# Autodesk Inventor assembly: Rotary_system_1
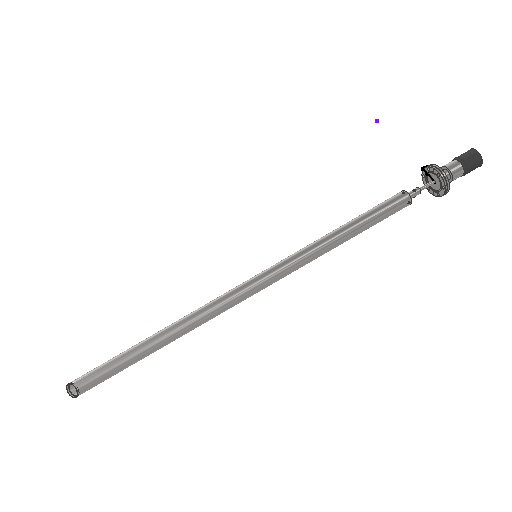
[picture p0: Inventor's stored thumbnail of the model, 512x512]
Saved by Autodesk Inventor 2026.2 (Build 302298000, 298)
## iProperties
Created: 2026-06-01
Part Number: Rotary_system_1
Document SubType Name: Assembly
Designer: zetsu
Author: zetsu
## Documents named in this file (7)
- D:\repos\PIHTI\BoronProbe_5\Figures\Rotary_system_1.iam
- D:\repos\PIHTI\BoronProbe_5\parts\B_probe_pipe_5.ipt
- D:\repos\PIHTI\BoronProbe_5\parts\rotary_transfer_shaft_5_1.ipt
- D:\repos\PIHTI\BoronProbe_5\parts\Rotary_Feedthrough\Rotary_Feedthrough.iam
- D:\repos\PIHTI\BoronProbe_5\parts\M3x10-BHCS.ipt
- D:\repos\PIHTI\BoronProbe_5\parts\M3x20-BHCS.ipt
- D:\repos\PIHTI\BoronProbe_5\parts\M3-nut.ipt
## Components (9 placed, 5 different names)
1. B_probe_pipe_5:1 — メイト:1, メイト:2, メイト:3, メイト:5, メイト:7, メイト:9
2. rotary_transfer_shaft_5_1:1 — メイト:1, メイト:2, メイト:4, メイト:6, メイト:8, メイト:10, メイト:11, メイト:12, メイト:13, メイト:14, メイト:15
3. Rotary_Feedthrough:1 [sub-assembly] — メイト:11, メイト:12
4. Broached Hexagon Socket Button Head Cap Screw - Metric M3 x 0.5 x 6:1 — メイト:3, メイト:4
5. Broached Hexagon Socket Button Head Cap Screw - Metric M3 x 0.5 x 6:2 — メイト:5, メイト:6
6. Broached Hexagon Socket Button Head Cap Screw - Metric M3 x 0.5 x 6:3 — メイト:7, メイト:8
7. Broached Hexagon Socket Button Head Cap Screw - Metric M3 x 0.5 x 6:4 — メイト:9, メイト:10
8. Broached Hexagon Socket Button Head Cap Screw - Metric M3 x 0.5 x 6:5 — メイト:13, メイト:14, メイト:16
9. JIS B 1181 Style 1 - Metric A M3:1 — メイト:15, メイト:16
## Relationships (16: Mate 16)
- メイト:1 [Mate]: B_probe_pipe_5:1 ↔ rotary_transfer_shaft_5_1:1
- メイト:2 [Mate]: B_probe_pipe_5:1 ↔ rotary_transfer_shaft_5_1:1
- メイト:3 [Mate]: B_probe_pipe_5:1 ↔ Broached Hexagon Socket Button Head Cap Screw - Metric M3 x 0.5 x 6:1
- メイト:4 [Mate]: rotary_transfer_shaft_5_1:1 ↔ Broached Hexagon Socket Button Head Cap Screw - Metric M3 x 0.5 x 6:1
- メイト:5 [Mate]: B_probe_pipe_5:1 ↔ Broached Hexagon Socket Button Head Cap Screw - Metric M3 x 0.5 x 6:2
- メイト:6 [Mate]: rotary_transfer_shaft_5_1:1 ↔ Broached Hexagon Socket Button Head Cap Screw - Metric M3 x 0.5 x 6:2
- メイト:7 [Mate]: B_probe_pipe_5:1 ↔ Broached Hexagon Socket Button Head Cap Screw - Metric M3 x 0.5 x 6:3
- メイト:8 [Mate]: rotary_transfer_shaft_5_1:1 ↔ Broached Hexagon Socket Button Head Cap Screw - Metric M3 x 0.5 x 6:3
- メイト:9 [Mate]: B_probe_pipe_5:1 ↔ Broached Hexagon Socket Button Head Cap Screw - Metric M3 x 0.5 x 6:4
- メイト:10 [Mate]: rotary_transfer_shaft_5_1:1 ↔ Broached Hexagon Socket Button Head Cap Screw - Metric M3 x 0.5 x 6:4
- メイト:11 [Mate]: rotary_transfer_shaft_5_1:1 ↔ Rotary_Feedthrough:1
- メイト:12 [Mate]: rotary_transfer_shaft_5_1:1 ↔ Rotary_Feedthrough:1
- メイト:13 [Mate]: rotary_transfer_shaft_5_1:1 ↔ Broached Hexagon Socket Button Head Cap Screw - Metric M3 x 0.5 x 6:5
- メイト:14 [Mate]: rotary_transfer_shaft_5_1:1 ↔ Broached Hexagon Socket Button Head Cap Screw - Metric M3 x 0.5 x 6:5
- メイト:15 [Mate]: rotary_transfer_shaft_5_1:1 ↔ JIS B 1181 Style 1 - Metric A M3:1
- メイト:16 [Mate]: Broached Hexagon Socket Button Head Cap Screw - Metric M3 x 0.5 x 6:5 ↔ JIS B 1181 Style 1 - Metric A M3:1
